# Autodesk Inventor assembly: Assembly1
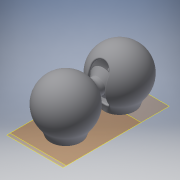
[picture p0: Inventor's stored thumbnail of the model, 180x180]
Saved by Autodesk Inventor 2017 (Build 210142000, 142)
## iProperties
Created: 2017-02-21
Part Number: Assembly1
Document SubType Name: Assembly
Designer: PLTW
Author: PLTW
## Documents named in this file (3)
- C:\Users\PLTW\Documents\Inventor\TeaCat\Assembly1.iam
- C:\Users\PLTW\Documents\Inventor\TeaCat\Body.ipt
- C:\Users\PLTW\Documents\Inventor\TeaCat\The Thing.ipt
## Components (2 placed, 2 different names)
1. Body:1 — Flush:1
2. The Thing:1 — Flush:1, Flush:2
## Relationships (2: Flush 2)
- Flush:1: Body:1 ↔ The Thing:1
- Flush:2: The Thing:1
